# Autodesk Inventor assembly: Outer Tie Rod
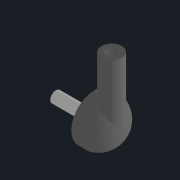
[picture p0: Inventor's stored thumbnail of the model, 180x180]
Saved by Autodesk Inventor 2021 (Build 250183000, 183)
## iProperties
Created: 2020-10-18
Part Number: Outer Tie Rod
Document SubType Name: Assembly
Designer: Eugene Tang
Mass: 57.3309 g
Surface Area: 189.837 cm^2
Volume: 57.3309 cm^3
Density: 1 g/cm^3
Author: Eugene Tang
## Documents named in this file (3)
- C:\Users\teuge\OneDrive - Curtin University of Technology Australia\Y4S2\DFM\Group Project\CAD\Master\Outer Tie Rod.iam
- C:\Users\teuge\OneDrive - Curtin University of Technology Australia\Y4S2\DFM\Group Project\CAD\Master\Outer Tie Rod.ipt
- C:\Users\teuge\OneDrive - Curtin University of Technology Australia\Y4S2\DFM\Group Project\CAD\Parts\Outer Tie Rod Ball.ipt
## Components (2 placed, 2 different names)
1. Outer Tie Rod:1
2. Outer Tie Rod Ball:1 — Flush:1
## Relationships (1: Flush 1)
- Flush:1: Outer Tie Rod Ball:1
